# Autodesk Inventor assembly: SYS-ASM-0000-Main
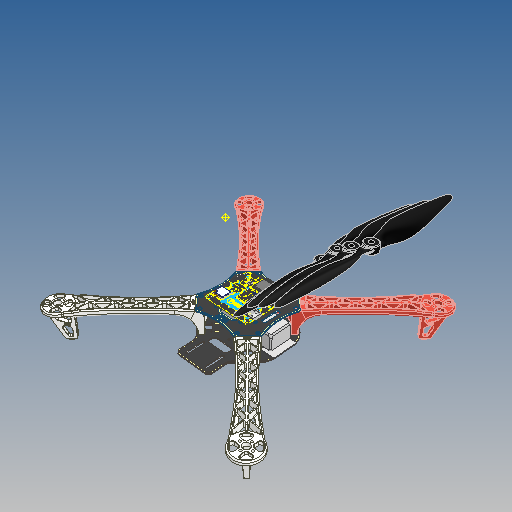
[picture p0: Inventor's stored thumbnail of the model, 512x512]
Saved by Autodesk Inventor 2026 (Build 300175000, 175)
## iProperties
Created: 2026-07-22
Part Number: SYS-ASM-0000-Main
Document SubType Name: Assembly
Designer: Pacman Ng
Author: Pacman Ng
## Documents named in this file (6)
- D:\OneDrive_MSFT\Work\Drone Research\3d_models\Full_body\SYS-ASM-0000-Main.iam
- D:\OneDrive_MSFT\Work\Drone Research\3d_models\Full_body\MEC-ASM-1000-F450_Frame.iam
- D:\OneDrive_MSFT\Work\Drone Research\3d_models\Full_body\ELE-PRT-3001-Dummy_Power_Monitor.ipt
- D:\OneDrive_MSFT\Work\Drone Research\3d_models\Full_body\PWR-PRT-2001-Lipo3S.ipt
- D:\OneDrive_MSFT\Work\Drone Research\3d_models\Full_body\ELE-ASM-4000-Flight_Controller.iam
- D:\OneDrive_MSFT\Work\Drone Research\3d_models\Full_body\AVI-PRT-5001-Propeller_10x45.ipt
## Components (8 placed, 5 different names)
1. MEC-ASM-1000-F450_Frame:1 [sub-assembly] — Flush:1
2. ELE-PRT-3001-Dummy_Power_Monitor:1 — Flush:1
3. PWR-PRT-2001-Lipo3S:1
4. ELE-ASM-4000-Flight_Controller:1 [sub-assembly]
5. AVI-PRT-5001-Propeller_10x45:1
6. AVI-PRT-5001-Propeller_10x45:2
7. AVI-PRT-5001-Propeller_10x45:3
8. AVI-PRT-5001-Propeller_10x45:4
## Relationships (1: Flush 1)
- Flush:1: MEC-ASM-1000-F450_Frame:1 ↔ ELE-PRT-3001-Dummy_Power_Monitor:1
